# Autodesk Inventor assembly: Assembly3
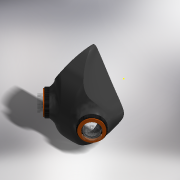
[picture p0: Inventor's stored thumbnail of the model, 180x180]
Saved by Autodesk Inventor 2021 (Build 250183000, 183)
## iProperties
Created: 2020-06-16
Part Number: Assembly3
Document SubType Name: Assembly
Designer: Derm
Author: Derm
## Documents named in this file (5)
- C:\Users\Derm\n95\v7\Assembly3.iam
- C:\Users\Derm\n95\v7\maskBodyV2.ipt
- C:\Users\Derm\n95\v7\3dpBayonetteMountV1Fastener.ipt
- C:\Users\Derm\n95\v7\3dpBayonetteMountV2.ipt
- C:\Users\Derm\n95\v7\outerMountGasket.ipt
## Components (7 placed, 4 different names)
1. maskBodyV2:1 — Mate:1, Mate:2, Mate:3, Mate:4, Mate:6, Mate:7
2. 3dpBayonetteMountV1Fastener:1 — Mate:5, Mate:6, Mate:9
3. 3dpBayonetteMountV2:1 — Mate:1, Mate:2, Mate:5, Mate:12
4. outerMountGasket:1 — Mate:9, Mate:12
5. 3dpBayonetteMountV1Fastener:2 — Mate:7, Mate:8, Mate:10
6. 3dpBayonetteMountV2:2 — Mate:3, Mate:4, Mate:8, Mate:11
7. outerMountGasket:2 — Mate:10, Mate:11
## Relationships (12: Mate 12)
- Mate:1: maskBodyV2:1 ↔ 3dpBayonetteMountV2:1
- Mate:2: maskBodyV2:1 ↔ 3dpBayonetteMountV2:1
- Mate:3: maskBodyV2:1 ↔ 3dpBayonetteMountV2:2
- Mate:4: maskBodyV2:1 ↔ 3dpBayonetteMountV2:2
- Mate:5: 3dpBayonetteMountV1Fastener:1 ↔ 3dpBayonetteMountV2:1
- Mate:6: maskBodyV2:1 ↔ 3dpBayonetteMountV1Fastener:1
- Mate:7: maskBodyV2:1 ↔ 3dpBayonetteMountV1Fastener:2
- Mate:8: 3dpBayonetteMountV1Fastener:2 ↔ 3dpBayonetteMountV2:2
- Mate:9: 3dpBayonetteMountV1Fastener:1 ↔ outerMountGasket:1
- Mate:10: 3dpBayonetteMountV1Fastener:2 ↔ outerMountGasket:2
- Mate:11: 3dpBayonetteMountV2:2 ↔ outerMountGasket:2
- Mate:12: 3dpBayonetteMountV2:1 ↔ outerMountGasket:1
